# Autodesk Inventor assembly: 悬架
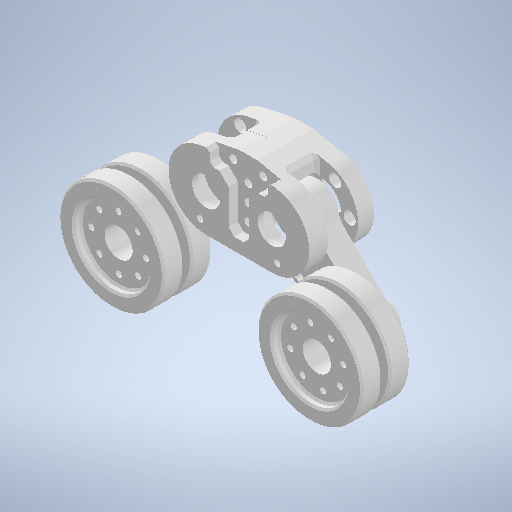
[picture p0: Inventor's stored thumbnail of the model, 512x512]
Saved by Autodesk Inventor 2025.1 (Build 291241000, 241)
## iProperties
Created: 2025-08-27
Part Number: 悬架
Document SubType Name: Assembly
Designer: Piw
Author: Piw
## Documents named in this file (6)
- C:\Users\22982\Desktop\急急急\Classis\悬架.iam
- C:\Users\22982\Desktop\急急急\Classis\悬臂架.ipt
- C:\Users\22982\Desktop\急急急\Classis\摇臂.ipt
- C:\Users\22982\Desktop\急急急\Classis\悬臂盖.ipt
- C:\Users\22982\Desktop\急急急\Classis\内轮.ipt
- C:\Users\22982\Desktop\急急急\Classis\外轮.ipt
## Components (8 placed, 5 different names)
1. 悬臂架:1 — 旋转:1, 配合:1, 配合:2, 旋转:4, 配合:11
2. 摇臂:1 — 旋转:1, 旋转:6
3. 悬臂盖:1 — 配合:1, 配合:2, 配合:11
4. 摇臂:2 — 旋转:4, 旋转:5
5. 内轮:2 — 旋转:5, 配合:7
6. 外轮:2 — 配合:7
7. 内轮:3 — 旋转:6
8. 外轮:3
## Relationships (13: Mate 9, RevoluteJoint 4)
- 旋转:1 [RevoluteJoint]: 悬臂架:1 ↔ 摇臂:1
- 配合:1 [Mate]: 悬臂架:1 ↔ 悬臂盖:1
- 配合:2 [Mate]: 悬臂架:1 ↔ 悬臂盖:1
- 旋转:4 [RevoluteJoint]: 悬臂架:1 ↔ 摇臂:2
- [Mate]: 内轮:2 ↔ 外轮:2
- [Mate]: 内轮:2 ↔ 外轮:2
- 旋转:5 [RevoluteJoint]: 摇臂:2 ↔ 内轮:2
- 配合:7 [Mate]: 内轮:2 ↔ 外轮:2
- [Mate]: 内轮:3 ↔ 外轮:3
- [Mate]: 内轮:3 ↔ 外轮:3
- [Mate]: 内轮:3 ↔ 外轮:3
- 配合:11 [Mate]: 悬臂架:1 ↔ 悬臂盖:1
- 旋转:6 [RevoluteJoint]: 摇臂:1 ↔ 内轮:3
## Named parameters: d28_d22 = 0 mm, d29_d23 = 0 mm, d33_d28_d22 = 0 mm, d34_d29_d23 = 0 mm, d35_d32 = 0 mm
